# Autodesk Inventor assembly: Сборка1
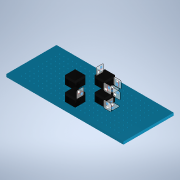
[picture p0: Inventor's stored thumbnail of the model, 180x180]
Saved by Autodesk Inventor 2022.3 (Build 263350000, 350)
## iProperties
Created: 2022-06-07
Part Number: Сборка1
Document SubType Name: Assembly
Designer: Admin
Author: Admin
## Documents named in this file (3)
- D:\папка для папок с папками\Проекты\Механизм кирилла\Проект хроматографического сборщика\Кнопки на плате.iam
- D:\папка для папок с папками\Проекты\Механизм кирилла\Проект хроматографического сборщика\плата панели.ipt
- D:\папка для папок с папками\Проекты\Механизм кирилла\Проект хроматографического сборщика\Кнопка маленькая.ipt
## Components (5 placed, 2 different names)
1. плата панели:1 — Совмещение:1, Совмещение:2, Совмещение:3, Совмещение:4, Заподлицо:7, Заподлицо:8
2. Кнопка маленькая:1 — Совмещение:1, Заподлицо:4, Совмещение:5
3. Кнопка маленькая:2 — Совмещение:2, Заподлицо:6, Совмещение:6, Совмещение:8, Совмещение:9, Заподлицо:7
4. Кнопка маленькая:3 — Совмещение:4, Заподлицо:6, Совмещение:6, Заподлицо:8
5. Кнопка маленькая:4 — Совмещение:3, Заподлицо:4, Совмещение:5, Совмещение:8, Совмещение:9
## Relationships (12: Mate 8, Flush 4)
- Совмещение:1 [Mate]: плата панели:1 ↔ Кнопка маленькая:1
- Совмещение:2 [Mate]: плата панели:1 ↔ Кнопка маленькая:2
- Совмещение:3 [Mate]: плата панели:1 ↔ Кнопка маленькая:4
- Совмещение:4 [Mate]: плата панели:1 ↔ Кнопка маленькая:3
- Заподлицо:4 [Flush]: Кнопка маленькая:1 ↔ Кнопка маленькая:4
- Заподлицо:6 [Flush]: Кнопка маленькая:2 ↔ Кнопка маленькая:3
- Совмещение:5 [Mate] (11.78 mm): Кнопка маленькая:1 ↔ Кнопка маленькая:4
- Совмещение:6 [Mate] (11.78 mm): Кнопка маленькая:2 ↔ Кнопка маленькая:3
- Совмещение:8 [Mate] (2.89 mm): Кнопка маленькая:2 ↔ Кнопка маленькая:4
- Совмещение:9 [Mate] (2.89 mm): Кнопка маленькая:2 ↔ Кнопка маленькая:4
- Заподлицо:7 [Flush] (3.11 mm): плата панели:1 ↔ Кнопка маленькая:2
- Заподлицо:8 [Flush] (-32 mm): плата панели:1 ↔ Кнопка маленькая:3
